# Autodesk Inventor assembly: SocketAssembly
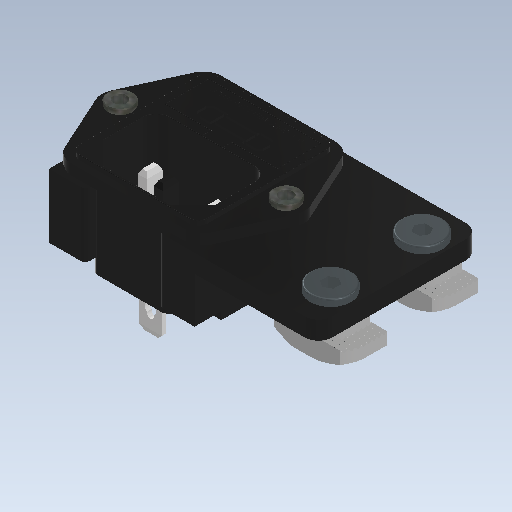
[picture p0: Inventor's stored thumbnail of the model, 512x512]
Saved by Autodesk Inventor 2020.2 (Build 242310000, 310)
## iProperties
Created: 2020-08-28
Part Number: SocketAssembly
Document SubType Name: Assembly
Designer: JK
Author: JK
## Documents named in this file (7)
- C:\Users\JK\Documents\Inventor\Anet Upgrade\SocketAssembly.iam
- C:\Users\JK\Documents\Inventor\Anet Upgrade\SocketMount.ipt
- C:\Users\JK\Documents\Inventor\Anet Upgrade\M5x12BoltFlatHead.ipt
- C:\Users\JK\Documents\Inventor\Anet Upgrade\T_Slot_Nut_Dropin_3030m5ipt.ipt
- C:\Users\JK\Documents\Inventor\Anet Upgrade\PowerInlet.ipt
- C:\Users\JK\Documents\Inventor\Anet Upgrade\M3Nut.ipt
- C:\Users\JK\Documents\Inventor\Anet Upgrade\M3x15Bolt.ipt
## Components (10 placed, 6 different names)
1. SocketMount:1
2. M5x12BoltFlatHead:1
3. M5x12BoltFlatHead:2
4. T_Slot_Nut_Dropin_3030m5ipt:1
5. T_Slot_Nut_Dropin_3030m5ipt:2
6. PowerInlet:1
7. M3Nut:1
8. M3Nut:2
9. M3x15Bolt:1
10. M3x15Bolt:2
## Relationships (22: Mate 14, Flush 5, Angle 3)
- [Mate]: SocketMount:1 ↔ M5x12BoltFlatHead:1
- [Mate]: SocketMount:1 ↔ M5x12BoltFlatHead:2
- [Mate]: M5x12BoltFlatHead:1 ↔ T_Slot_Nut_Dropin_3030m5ipt:1
- [Mate]: M5x12BoltFlatHead:2 ↔ T_Slot_Nut_Dropin_3030m5ipt:2
- [Flush]: M5x12BoltFlatHead:1 ↔ M5x12BoltFlatHead:2
- [Mate]: SocketMount:1 ↔ M5x12BoltFlatHead:1
- [Mate]: SocketMount:1 ↔ T_Slot_Nut_Dropin_3030m5ipt:1
- [Flush]: T_Slot_Nut_Dropin_3030m5ipt:1 ↔ T_Slot_Nut_Dropin_3030m5ipt:2
- [Angle] (0 deg): SocketMount:1 ↔ T_Slot_Nut_Dropin_3030m5ipt:1
- [Angle] (0 deg): T_Slot_Nut_Dropin_3030m5ipt:1 ↔ T_Slot_Nut_Dropin_3030m5ipt:2
- [Mate]: SocketMount:1 ↔ PowerInlet:1
- [Mate]: SocketMount:1 ↔ PowerInlet:1
- [Angle] (0 deg): SocketMount:1 ↔ PowerInlet:1
- [Mate]: PowerInlet:1 ↔ M3x15Bolt:1
- [Mate]: PowerInlet:1 ↔ M3x15Bolt:2
- [Flush]: M3x15Bolt:1 ↔ M3x15Bolt:2
- [Mate]: M3Nut:1 ↔ M3x15Bolt:1
- [Mate]: M3Nut:2 ↔ M3x15Bolt:2
- [Mate]: PowerInlet:1 ↔ M3x15Bolt:2
- [Flush]: M3x15Bolt:1 ↔ M3x15Bolt:2
- [Mate]: SocketMount:1 ↔ M3Nut:2
- [Flush]: M3Nut:1 ↔ M3Nut:2
